# Autodesk Inventor assembly: TSI_Assembly
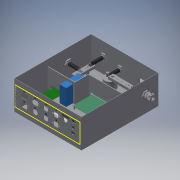
[picture p0: Inventor's stored thumbnail of the model, 180x180]
Saved by Autodesk Inventor 2017 (Build 210142000, 142)
## iProperties
Created: 2017-02-28
Part Number: TSI_Assembly
Document SubType Name: Assembly
Designer: Christer Hoeflinger
Author: Christer Hoeflinger
## Documents named in this file (23)
- P:\me_fsae\Independent Study Battery Pack Deliverables\2016 Inventor Model - Copy\2016 Directory\Electrical\TSI Box\From Chris 2\TSI_Assembly.iam
- P:\me_fsae\Independent Study Battery Pack Deliverables\2016 Inventor Model - Copy\2016 Directory\Electrical\TSI Box\From Chris 2\15x11Plate.ipt
- P:\me_fsae\Independent Study Battery Pack Deliverables\2016 Inventor Model - Copy\2016 Directory\Electrical\TSI Box\From Chris 2\IMD20216.ipt
- P:\me_fsae\Independent Study Battery Pack Deliverables\2016 Inventor Model - Copy\2016 Directory\Electrical\TSI Box\From Chris 2\PrechargeRelay2016.ipt
- P:\me_fsae\Independent Study Battery Pack Deliverables\2016 Inventor Model - Copy\2016 Directory\Electrical\TSI Box\From Chris 2\18x12x6Box.ipt
- P:\me_fsae\Independent Study Battery Pack Deliverables\2016 Inventor Model - Copy\2016 Directory\Electrical\TSI Box\From Chris 2\L16-TSV-65.1.iam
- P:\me_fsae\Independent Study Battery Pack Deliverables\2016 Inventor Model - Copy\2016 Directory\Electrical\TSI Box\From Chris 2\Current Sensor Bar.ipt
- P:\me_fsae\Independent Study Battery Pack Deliverables\2016 Inventor Model - Copy\2016 Directory\Electrical\TSI Box\From Chris 2\MockPCB.ipt
- P:\me_fsae\Independent Study Battery Pack Deliverables\2016 Inventor Model - Copy\2016 Directory\Electrical\TSI Box\From Chris 2\Ring Connector model 3.ipt
- P:\me_fsae\Independent Study Battery Pack Deliverables\2016 Inventor Model - Copy\2016 Directory\Electrical\TSI Box\From Chris 2\CAN2CAN.ipt
- P:\me_fsae\Independent Study Battery Pack Deliverables\2016 Inventor Model - Copy\2016 Directory\Electrical\TSI Box\From Chris 2\BackPanel.ipt
- P:\me_fsae\Independent Study Battery Pack Deliverables\2016 Inventor Model - Copy\2016 Directory\Electrical\TSI Box\From Chris 2\TSV-Bar.ipt
- P:\me_fsae\Independent Study Battery Pack Deliverables\2016 Inventor Model - Copy\2016 Directory\Electrical\TSI Box\From Chris 2\FrontPanel.ipt
- P:\me_fsae\Independent Study Battery Pack Deliverables\2016 Inventor Model - Copy\2016 Directory\Electrical\TSI Box\From Chris 2\DIN Rail (TS) 35mm Wide v1\TS35x7.5 mm H - 5.2 mm dia slot - 100 mm long.ipt
- P:\me_fsae\Independent Study Battery Pack Deliverables\2016 Inventor Model - Copy\2016 Directory\Electrical\TSI Box\From Chris 2\DIN Rail (TS) 35mm Wide v1.ipt
- P:\me_fsae\Independent Study Battery Pack Deliverables\2016 Inventor Model - Copy\2016 Directory\Electrical\TSI Box\From Chris 2\CANIMDWall.ipt
- P:\me_fsae\Independent Study Battery Pack Deliverables\2016 Inventor Model - Copy\2016 Directory\Electrical\TSI Box\From Chris 2\WallBend.ipt
- P:\me_fsae\Independent Study Battery Pack Deliverables\2016 Inventor Model - Copy\2016 Directory\Electrical\TSI Box\From Chris 2\PCBWall.ipt
- P:\me_fsae\Independent Study Battery Pack Deliverables\2016 Inventor Model - Copy\2016 Directory\Electrical\TSI Box\From Chris 2\2inchMcMasterStandoff.ipt
- P:\me_fsae\Independent Study Battery Pack Deliverables\2016 Inventor Model - Copy\2016 Directory\Electrical\TSI Box\From Chris 2\94335A115_ELECTRICAL-INSULATING FEM THRDED STANDOFF.ipt
- P:\me_fsae\Independent Study Battery Pack Deliverables\2016 Inventor Model - Copy\2016 Directory\Electrical\TSI Box\From Chris 2\6-32 .25 inch screw.ipt
- P:\me_fsae\Independent Study Battery Pack Deliverables\2016 Inventor Model - Copy\2016 Directory\Electrical\TSI Box\From Chris 2\6-32 inserts.ipt
- P:\me_fsae\Independent Study Battery Pack Deliverables\2016 Inventor Model - Copy\2016 Directory\Electrical\TSI Box\From Chris 2\1 inch screw.ipt
## Components (66 placed, 21 different names)
1. 15x11Plate:1 — Mate:3, Mate:19, Flush:25, Flush:26, Mate:26, Mate:28, Mate:29, Flush:29, Flush:30, Mate:35, Mate:41, Mate:43, Mate:45, Mate:49, Insert:47, Insert:48, Insert:49, Insert:50, Insert:51, Insert:52, Insert:53, Insert:54, Insert:55, Insert:56, Insert:57, Insert:58, Insert:69, Insert:70, Insert:71, Insert:72, Insert:73, Insert:74, Insert:75, Insert:76, Insert:77, Insert:78, Insert:79, Insert:80, Insert:81, Insert:82, Insert:83, Insert:84, Insert:85, Angle:36
2. 18x12x6Box:1 — Mate:3, Angle:1, Angle:12, Insert:26, Angle:23, Insert:29, Insert:31, Angle:25, Flush:25, Flush:26, Angle:27, Angle:28, Angle:29, Insert:37, Angle:30, Mate:30, Flush:27, Flush:28, Flush:42, Insert:41, Insert:42, Mate:42, Mate:48
3. L16-TSV-65.1:1 [sub-assembly] — Angle:1, Insert:29, Insert:35
4. L16-TSV-65.1:4 [sub-assembly] — Insert:20, Insert:31, Angle:25
5. Ring Connector model 3:1 — Angle:12, Insert:20, Mate:27
6. Ring Connector model 3:2 — Insert:27, Angle:36
7. IMD20216:2 — Mate:19, Flush:30, Mate:31, Insert:63, Insert:64, Insert:65, Insert:66, Insert:67, Insert:68
8. CAN2CAN:1 — Mate:29, Mate:31, Mate:47
9. L16-TSV-65.1:5 [sub-assembly] — Insert:26, Angle:23, Insert:27
10. MockPCB:1 — Mate:26, Angle:28, Flush:29, Flush:42, Flush:51, Insert:59, Insert:60, Insert:61, Insert:62
11. PrechargeRelay2016:1 — Mate:27, Mate:28, Angle:27, Insert:43
12. Ring Connector model 3:3 — Insert:89
13. Ring Connector model 3:4 — Insert:35, Angle:29
14. L16-TSV-65.1:6 [sub-assembly] — Insert:37, Angle:30
15. FrontPanel:1 — Mate:30, Flush:27, Flush:28
16. TS35x7.5 mm H - 5.2 mm dia slot - 100 mm long:1 — Mate:35, Mate:47, Mate:48, Mate:50, Flush:50
17. TSV-Bar:2 — Insert:86, Insert:87, Insert:89
18. BackPanel:1 — Insert:41, Insert:42, Angle:35
19. CANIMDWall:1 — Mate:41, Mate:42, Mate:44, Flush:48
20. WallBend:1 — Mate:43, Mate:44, Flush:48, Mate:46, Flush:49
21. PCBWall:1 — Mate:45, Mate:46, Flush:49, Flush:51
22. Current Sensor Bar:1 — Insert:43, Angle:35, Insert:88
23. 2inchMcMasterStandoff:1 — Insert:47
24. 2inchMcMasterStandoff:2
25. 2inchMcMasterStandoff:3 — Insert:48
26. TS35x7.5 mm H - 5.2 mm dia slot - 100 mm long:2 — Mate:49, Mate:50, Flush:50
27. 94335A115_ELECTRICAL-INSULATING FEM THRDED STANDOFF:1 — Insert:53
28. 94335A115_ELECTRICAL-INSULATING FEM THRDED STANDOFF:2 — Insert:54
29. 94335A115_ELECTRICAL-INSULATING FEM THRDED STANDOFF:3 — Insert:55
30. 94335A115_ELECTRICAL-INSULATING FEM THRDED STANDOFF:4 — Insert:56
31. 94335A115_ELECTRICAL-INSULATING FEM THRDED STANDOFF:5 — Insert:57
32. 94335A115_ELECTRICAL-INSULATING FEM THRDED STANDOFF:6 — Insert:58
33. 94335A115_ELECTRICAL-INSULATING FEM THRDED STANDOFF:7 — Insert:51
34. 94335A115_ELECTRICAL-INSULATING FEM THRDED STANDOFF:8 — Insert:52
35. 94335A115_ELECTRICAL-INSULATING FEM THRDED STANDOFF:9 — Insert:50
36. 94335A115_ELECTRICAL-INSULATING FEM THRDED STANDOFF:10 — Insert:49
37. 6-32 .25 inch screw:1 — Insert:68
38. 6-32 .25 inch screw:2 — Insert:67
39. 6-32 .25 inch screw:3 — Insert:64
40. 6-32 .25 inch screw:4 — Insert:66
41. 6-32 .25 inch screw:5 — Insert:63
42. 6-32 .25 inch screw:6 — Insert:65
43. 6-32 .25 inch screw:7 — Insert:60
44. 6-32 .25 inch screw:8 — Insert:59
45. 6-32 .25 inch screw:9 — Insert:61
46. 6-32 .25 inch screw:10 — Insert:62
47. 6-32 inserts:1 — Insert:81
48. 6-32 inserts:2 — Insert:80
49. 6-32 inserts:3 — Insert:79
50. 6-32 inserts:4 — Insert:76
51. 6-32 inserts:5 — Insert:78
52. 6-32 inserts:6 — Insert:77
53. 6-32 inserts:7 — Insert:73
54. 6-32 inserts:8 — Insert:71
55. 6-32 inserts:9 — Insert:74
56. 6-32 inserts:10 — Insert:72
57. 6-32 inserts:11 — Insert:83
58. 6-32 inserts:12 — Insert:82
59. 6-32 inserts:13 — Insert:75
60. 6-32 inserts:14 — Insert:70
61. 6-32 inserts:15 — Insert:69
62. 6-32 .25 inch screw:11 — Insert:84
63. 6-32 .25 inch screw:12 — Insert:85
64. 1 inch screw:1 — Insert:86
65. 1 inch screw:2 — Insert:87
66. 1 inch screw:3 — Insert:88
## Relationships (93: Insert 53, Mate 19, Flush 11, Angle 10)
- Mate:3 (11.1125 mm): 15x11Plate:1 ↔ 18x12x6Box:1
- Angle:1 (0 deg): 18x12x6Box:1 ↔ L16-TSV-65.1:1
- Angle:12 (180 deg): 18x12x6Box:1 ↔ Ring Connector model 3:1
- Insert:20: L16-TSV-65.1:4 ↔ Ring Connector model 3:1
- Mate:19 (12.7 mm): 15x11Plate:1 ↔ IMD20216:2
- Insert:26: 18x12x6Box:1 ↔ L16-TSV-65.1:5
- Angle:23 (0 deg): 18x12x6Box:1 ↔ L16-TSV-65.1:5
- Insert:27: Ring Connector model 3:2 ↔ L16-TSV-65.1:5
- Insert:29: 18x12x6Box:1 ↔ L16-TSV-65.1:1
- Insert:31: 18x12x6Box:1 ↔ L16-TSV-65.1:4
- Angle:25 (0 deg): 18x12x6Box:1 ↔ L16-TSV-65.1:4
- Flush:25 (14.2875 mm): 15x11Plate:1 ↔ 18x12x6Box:1
- Flush:26 (15.875 mm): 15x11Plate:1 ↔ 18x12x6Box:1
- Mate:26 (12.7 mm): 15x11Plate:1 ↔ MockPCB:1
- Mate:27: Ring Connector model 3:1 ↔ PrechargeRelay2016:1
- Mate:28: 15x11Plate:1 ↔ PrechargeRelay2016:1
- Angle:27 (180 deg): 18x12x6Box:1 ↔ PrechargeRelay2016:1
- Mate:29: 15x11Plate:1 ↔ CAN2CAN:1
- Angle:28 (0 deg): 18x12x6Box:1 ↔ MockPCB:1
- Insert:35: L16-TSV-65.1:1 ↔ Ring Connector model 3:4
- Angle:29 (0 deg): 18x12x6Box:1 ↔ Ring Connector model 3:4
- Insert:37: 18x12x6Box:1 ↔ L16-TSV-65.1:6
- Angle:30 (0 deg): 18x12x6Box:1 ↔ L16-TSV-65.1:6
- Mate:30: 18x12x6Box:1 ↔ FrontPanel:1
- Flush:27 (6.35 mm): 18x12x6Box:1 ↔ FrontPanel:1
- Flush:28 (-25.4 mm): 18x12x6Box:1 ↔ FrontPanel:1
- Flush:29 (6.35 mm): 15x11Plate:1 ↔ MockPCB:1
- Flush:30 (6.35 mm): 15x11Plate:1 ↔ IMD20216:2
- Mate:31 (19.05 mm): IMD20216:2 ↔ CAN2CAN:1
- Mate:35: 15x11Plate:1 ↔ TS35x7.5 mm H - 5.2 mm dia slot - 100 mm long:1
- Flush:42 (-254 mm): 18x12x6Box:1 ↔ MockPCB:1
- Insert:41: 18x12x6Box:1 ↔ BackPanel:1
- Insert:42: 18x12x6Box:1 ↔ BackPanel:1
- Mate:41: 15x11Plate:1 ↔ CANIMDWall:1
- Mate:42: 18x12x6Box:1 ↔ CANIMDWall:1
- Mate:43: 15x11Plate:1 ↔ WallBend:1
- Mate:44: CANIMDWall:1 ↔ WallBend:1
- Flush:48: CANIMDWall:1 ↔ WallBend:1
- Mate:45: 15x11Plate:1 ↔ PCBWall:1
- Mate:46: WallBend:1 ↔ PCBWall:1
- Flush:49: WallBend:1 ↔ PCBWall:1
- Insert:43: PrechargeRelay2016:1 ↔ Current Sensor Bar:1
- Angle:35 (0 deg): BackPanel:1 ↔ Current Sensor Bar:1
- Mate:47 (50.8 mm): CAN2CAN:1 ↔ TS35x7.5 mm H - 5.2 mm dia slot - 100 mm long:1
- Mate:48 (25.4 mm): 18x12x6Box:1 ↔ TS35x7.5 mm H - 5.2 mm dia slot - 100 mm long:1
- Mate:49: 15x11Plate:1 ↔ TS35x7.5 mm H - 5.2 mm dia slot - 100 mm long:2
- Mate:50: TS35x7.5 mm H - 5.2 mm dia slot - 100 mm long:1 ↔ TS35x7.5 mm H - 5.2 mm dia slot - 100 mm long:2
- Flush:50: TS35x7.5 mm H - 5.2 mm dia slot - 100 mm long:1 ↔ TS35x7.5 mm H - 5.2 mm dia slot - 100 mm long:2
- Insert:47: 15x11Plate:1 ↔ 2inchMcMasterStandoff:1
- Insert:48: 15x11Plate:1 ↔ 2inchMcMasterStandoff:3
- Flush:51: MockPCB:1 ↔ PCBWall:1
- Insert:49: 15x11Plate:1 ↔ 94335A115_ELECTRICAL-INSULATING FEM THRDED STANDOFF:10
- Insert:50: 15x11Plate:1 ↔ 94335A115_ELECTRICAL-INSULATING FEM THRDED STANDOFF:9
- Insert:51: 15x11Plate:1 ↔ 94335A115_ELECTRICAL-INSULATING FEM THRDED STANDOFF:7
- Insert:52: 15x11Plate:1 ↔ 94335A115_ELECTRICAL-INSULATING FEM THRDED STANDOFF:8
- Insert:53: 15x11Plate:1 ↔ 94335A115_ELECTRICAL-INSULATING FEM THRDED STANDOFF:1
- Insert:54: 15x11Plate:1 ↔ 94335A115_ELECTRICAL-INSULATING FEM THRDED STANDOFF:2
- Insert:55: 15x11Plate:1 ↔ 94335A115_ELECTRICAL-INSULATING FEM THRDED STANDOFF:3
- Insert:56: 15x11Plate:1 ↔ 94335A115_ELECTRICAL-INSULATING FEM THRDED STANDOFF:4
- Insert:57: 15x11Plate:1 ↔ 94335A115_ELECTRICAL-INSULATING FEM THRDED STANDOFF:5
- Insert:58: 15x11Plate:1 ↔ 94335A115_ELECTRICAL-INSULATING FEM THRDED STANDOFF:6
- Insert:59: MockPCB:1 ↔ 6-32 .25 inch screw:8
- Insert:60: MockPCB:1 ↔ 6-32 .25 inch screw:7
- Insert:61: MockPCB:1 ↔ 6-32 .25 inch screw:9
- Insert:62: MockPCB:1 ↔ 6-32 .25 inch screw:10
- Insert:63: IMD20216:2 ↔ 6-32 .25 inch screw:5
- Insert:64: IMD20216:2 ↔ 6-32 .25 inch screw:3
- Insert:65: IMD20216:2 ↔ 6-32 .25 inch screw:6
- Insert:66: IMD20216:2 ↔ 6-32 .25 inch screw:4
- Insert:67: IMD20216:2 ↔ 6-32 .25 inch screw:2
- Insert:68: IMD20216:2 ↔ 6-32 .25 inch screw:1
- Insert:69: 15x11Plate:1 ↔ 6-32 inserts:15
- Insert:70: 15x11Plate:1 ↔ 6-32 inserts:14
- Insert:71: 15x11Plate:1 ↔ 6-32 inserts:8
- Insert:72: 15x11Plate:1 ↔ 6-32 inserts:10
- Insert:73: 15x11Plate:1 ↔ 6-32 inserts:7
- Insert:74: 15x11Plate:1 ↔ 6-32 inserts:9
- Insert:75: 15x11Plate:1 ↔ 6-32 inserts:13
- Insert:76: 15x11Plate:1 ↔ 6-32 inserts:4
- Insert:77: 15x11Plate:1 ↔ 6-32 inserts:6
- Insert:78: 15x11Plate:1 ↔ 6-32 inserts:5
- Insert:79: 15x11Plate:1 ↔ 6-32 inserts:3
- Insert:80: 15x11Plate:1 ↔ 6-32 inserts:2
- Insert:81: 15x11Plate:1 ↔ 6-32 inserts:1
- Insert:82: 15x11Plate:1 ↔ 6-32 inserts:12
- Insert:83: 15x11Plate:1 ↔ 6-32 inserts:11
- Insert:84 (0.9906 mm): 15x11Plate:1 ↔ 6-32 .25 inch screw:11
- Insert:85 (0.9906 mm): 15x11Plate:1 ↔ 6-32 .25 inch screw:12
- Insert:86: TSV-Bar:2 ↔ 1 inch screw:1
- Insert:87: TSV-Bar:2 ↔ 1 inch screw:2
- Insert:88: Current Sensor Bar:1 ↔ 1 inch screw:3
- Insert:89: Ring Connector model 3:3 ↔ TSV-Bar:2
- Angle:36 (0 deg): 15x11Plate:1 ↔ Ring Connector model 3:2
